# Autodesk Inventor assembly: TKC
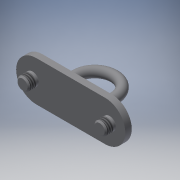
[picture p0: Inventor's stored thumbnail of the model, 180x180]
Saved by Autodesk Inventor 2019 (Build 230136000, 136)
## iProperties
Category: PARTsolutions
Company: MISUMI
Created: 2024-03-12
Part Number: TKC
Catalog Web Link: www.cadenas.de
Description: TKC-Mounting Brackets
Vendor: MISUMI
Document SubType Name: Assembly
Designer: psAdmin
Manufacturer: MISUMI
Mass: 1.05548 g
Surface Area: 15.4609 cm^2
Volume: 1.05548 cm^3
Density: 1 g/cm^3
Title: TKC
Author: Cadenas PARTsolutions
Comments: Mounting Brackets
PSOL_IDENT_0: {$CADENAS_DATA/23d-libs/misumi/metric/28_keys_magnets/tkc_asmtab.prj},157 {VTYP=3D},{STYP=ASSTAB},{N
PSOL_IDENT_1: B=TKC},{LINA=TKC},{NN=TKC},{DATE=17.03.2023 10:24:11},{GEOMDATE=17.03.2023 08:45:37},{VERSION=},{LIN
PSOL_IDENT_2: EID=10},{WBVAR=},{WBNUMERIC=}  {NB=TKC},{LINA=TKC},{KT=DUMMY},{PN=TKC},{TP=TKC},{MAT=304 Stainless S
PSOL_IDENT_3: teel},{AC=M4-5 Flat Head Screw (2 pcs.)},{MATAC=304 Stainless Steel},{RWL=20},{PPATH=tkc_asmtpl.prj}
NB: TKC
NN: TKC
NT: Mounting Brackets
NBSYN: $PN.
LINA: TKC
CATALOG: Misumi
PN: TKC
TP: TKC
SUPPLIER: MISUMI
ARTICLENO: TKC
BOMINFO: TKC
CREATOR: CADENAS GmbH
## Documents named in this file (3)
- e:\temp\worker_COMMON_4\temp\tmp_7628_144_zOlhd\format_0\TKC.iam
- e:\temp\worker_COMMON_4\temp\tmp_7628_144_zOlhd\format_0\TKCb.ipt
- e:\temp\worker_COMMON_4\temp\tmp_7628_144_zOlhd\format_0\FBb4-5.ipt
## Components (3 placed, 2 different names)
1. TKCb:1 — cp1_XY@1 <-> screw_XY@2, cp1_Z@1 <-> screw_Z@2, cp1_YZ@1 <-> screw_YZ@2, cp2_XY@1 <-> screw_XY@3, cp2_Z@1 <-> screw_Z@3, cp2_YZ@1 <-> screw_YZ@3
2. FBb4-5:1 — cp1_XY@1 <-> screw_XY@2, cp1_Z@1 <-> screw_Z@2, cp1_YZ@1 <-> screw_YZ@2
3. FBb4-5:2 — cp2_XY@1 <-> screw_XY@3, cp2_Z@1 <-> screw_Z@3, cp2_YZ@1 <-> screw_YZ@3
## Relationships (6: Mate 4, Angle 2)
- cp1_XY@1 <-> screw_XY@2 [Mate]: TKCb:1 ↔ FBb4-5:1
- cp1_Z@1 <-> screw_Z@2 [Mate]: TKCb:1 ↔ FBb4-5:1
- cp1_YZ@1 <-> screw_YZ@2 [Angle] (0 deg): TKCb:1 ↔ FBb4-5:1
- cp2_XY@1 <-> screw_XY@3 [Mate]: TKCb:1 ↔ FBb4-5:2
- cp2_Z@1 <-> screw_Z@3 [Mate]: TKCb:1 ↔ FBb4-5:2
- cp2_YZ@1 <-> screw_YZ@3 [Angle] (0 deg): TKCb:1 ↔ FBb4-5:2
